# Autodesk Inventor assembly: completely
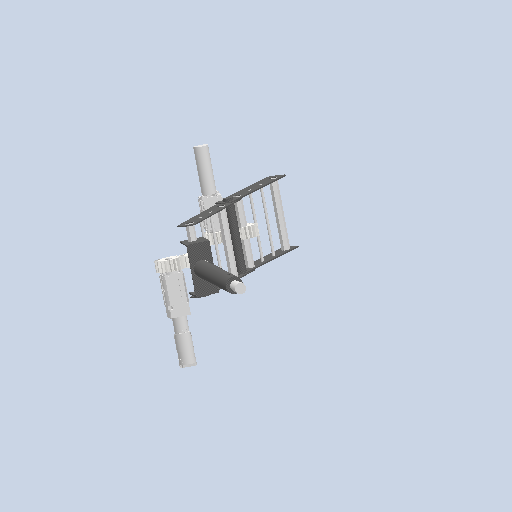
[picture p0: Inventor's stored thumbnail of the model, 512x512]
Saved by Autodesk Inventor 2023 (Build 270158000, 158)
## iProperties
Created: 2023-01-03
Part Number: completely
Document SubType Name: Assembly
Designer: victo
Author: victo
## Documents named in this file (11)
- C:\Users\victo\OneDrive\Documents\rcr\completely new\up to forearm full assembly.iam
- C:\Users\victo\OneDrive\Documents\rcr\completely new\arm one.iam
- C:\Users\victo\OneDrive\Documents\rcr\completely new\arm two.iam
- C:\Users\victo\OneDrive\Documents\rcr\completely new\Shaft connecting chass.ipt
- C:\Users\victo\OneDrive\Documents\rcr\completely new\shaft to bicep.ipt
- C:\Users\victo\OneDrive\Documents\rcr\completely new\econ gear.ipt
- C:\Users\victo\OneDrive\Documents\rcr\completely new\planetary motor.ipt
- C:\Users\victo\OneDrive\Documents\rcr\completely new\fg 3 Stage HD - 57 Sport (2).iam
- C:\Users\victo\OneDrive\Documents\rcr\completely new\bicep gearbox 1.iam
- C:\Users\victo\OneDrive\Documents\rcr\completely new\bicep motor.ipt
- C:\Users\victo\OneDrive\Documents\rcr\completely new\gear.iam
## Components (11 placed, 10 different names)
1. arm one:2 [sub-assembly] — Rotational:1, Angle:1, Mate:1, Mate:2, Flush:1, Mate:3, Rigid:6
2. arm two:1 [sub-assembly] — Rotational:1, Rigid:4
3. Shaft connecting chass:1 — Rigid:1, Rotational:2
4. shaft to bicep:1 — Angle:1, Mate:1, Mate:2, Flush:1, Mate:3, Rigid:1
5. econ gear:1 — Rotational:2
6. planetary motor:1 — Rigid:2
7. fg 3 Stage HD - 57 Sport (2):1 [sub-assembly] — Rigid:2, Rigid:5
8. bicep gearbox:1 [sub-assembly] — Rigid:3, Rigid:7
9. bicep motor:1 — Rigid:3
10. gear:1 [sub-assembly] — Rigid:6, Rigid:7
11. gear:2 [sub-assembly] — Rigid:4, Rigid:5
## Relationships (14: WeldJoint 7, Mate 3, RevoluteJoint 2, Angle 1, Flush 1)
- Rotational:1 [RevoluteJoint]: arm one:2 ↔ arm two:1
- Angle:1 (0 deg): arm one:2 ↔ shaft to bicep:1
- Mate:1: arm one:2 ↔ shaft to bicep:1
- Mate:2: arm one:2 ↔ shaft to bicep:1
- Flush:1 (6.35 mm): arm one:2 ↔ shaft to bicep:1
- Mate:3: arm one:2 ↔ shaft to bicep:1
- Rigid:1 [WeldJoint] (-6.35 mm): Shaft connecting chass:1 ↔ shaft to bicep:1
- Rotational:2 [RevoluteJoint]: Shaft connecting chass:1 ↔ econ gear:1
- Rigid:2 [WeldJoint]: planetary motor:1 ↔ fg 3 Stage HD - 57 Sport (2):1
- Rigid:3 [WeldJoint]: bicep gearbox:1 ↔ bicep motor:1
- Rigid:4 [WeldJoint]: arm two:1 ↔ gear:2
- Rigid:5 [WeldJoint]: fg 3 Stage HD - 57 Sport (2):1 ↔ gear:2
- Rigid:6 [WeldJoint]: arm one:2 ↔ gear:1
- Rigid:7 [WeldJoint]: bicep gearbox:1 ↔ gear:1
